# Autodesk Inventor assembly: FrameV4
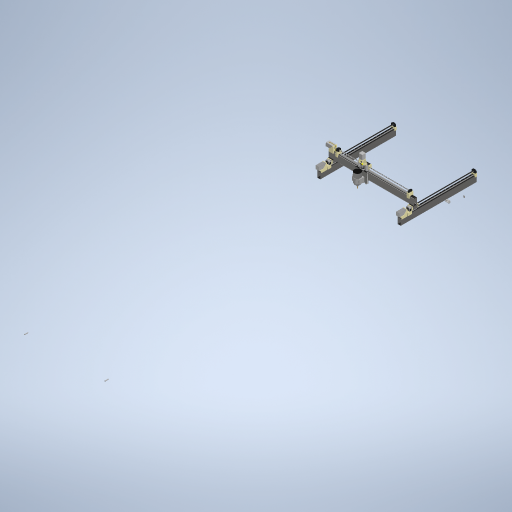
[picture p0: Inventor's stored thumbnail of the model, 512x512]
Saved by Autodesk Inventor 2023 (Build 270158000, 158)
## iProperties
Created: 2022-05-07
Part Number: FrameV4
Document SubType Name: Assembly
Designer: plebbb
Mass: 10930.1 g
Surface Area: 33660.3 cm^2
Volume: 10930.1 cm^3
Density: 1 g/cm^3
Author: plebbb
## Documents named in this file (27)
- C:\Users\a laptop\Desktop\CNC_Project\FrameV4.iam
- C:\Users\a laptop\Desktop\CNC_Project\Ballscrew_Assembly.iam
- C:\Users\a laptop\Desktop\CNC_Project\2x4_Tube.ipt
- C:\Users\a laptop\Desktop\CNC_Project\HGW20CC_Rail_800mm.ipt
- C:\Users\a laptop\Desktop\CNC_Project\BK10.ipt
- C:\Users\a laptop\Desktop\CNC_Project\BF10.ipt
- C:\Users\a laptop\Desktop\CNC_Project\Ballscrew_Assembly_1204.iam
- C:\Users\a laptop\Desktop\CNC_Project\SFU1204-500.ipt
- C:\Users\a laptop\Desktop\CNC_Project\BF10_Spacer.ipt
- C:\Users\a laptop\Desktop\CNC_Project\BK10_Spacer.ipt
- C:\Users\a laptop\Desktop\CNC_Project\2x3_L_Bracket.ipt
- C:\Users\a laptop\Desktop\CNC_Project\HGW20CC_Slider.ipt
- C:\Users\a laptop\Desktop\CNC_Project\HGW20CC_Rail_300mm.ipt
- C:\Users\a laptop\Desktop\CNC_Project\Z_PLATE.iam
- C:\Users\a laptop\Desktop\CNC_Project\SFU1204-300.ipt
- C:\Users\a laptop\Desktop\CNC_Project\Spindle.ipt
- C:\Users\a laptop\Desktop\CNC_Project\Drill_Bit.ipt
- C:\Users\a laptop\Desktop\CNC_Project\X_GANTRY.iam
- C:\Users\a laptop\Desktop\CNC_Project\Z_Gantry_Plate_Spaced.iam
- C:\Users\a laptop\Desktop\CNC_Project\Nema23.ipt
- C:\Users\a laptop\Desktop\CNC_Project\Nema23_Mount_short.ipt
- C:\Users\a laptop\Desktop\CNC_Project\SFU1204_Nut.ipt
- C:\Users\a laptop\Desktop\CNC_Project\DSG12H.ipt
- C:\Users\a laptop\Desktop\CNC_Project\Z_Motor_Holder.ipt
- C:\Users\a laptop\Desktop\CNC_Project\Nema23_Short.ipt
- C:\Users\a laptop\Desktop\CNC_Project\Xgantry_CableChain_bottom_connector.ipt
- C:\Users\a laptop\Desktop\CNC_Project\Xgantry_CableChain_top_connector.ipt
## Components (32 placed, 26 different names)
1. Ballscrew_Assembly:1 [sub-assembly] — Mate:7, Mate:8, Mate:11, Mate:84
2. Ballscrew_Assembly:2 [sub-assembly] — Mate:9, Mate:10, Mate:12, Mate:83, Mate:85, Mate:86
3. 2x4_Tube:1 — Mate:7, Mate:8, Mate:9, Mate:10, Mate:11, Mate:12, Flush:4, Mate:15, Mate:26, Mate:27, Mate:34, Mate:35, Flush:5, Mate:45
4. HGW20CC_Rail_800mm:1 — Flush:4, Mate:15, Mate:22, Mate:23, Mate:38, Flush:6, Flush:7
5. BK10:1 — Mate:40, Mate:41, Mate:42, Mate:43, Mate:44
6. BF10:1 — Mate:31, Mate:32, Mate:33, Mate:36
7. Ballscrew_Assembly_1204:1 [sub-assembly] — Mate:22, Mate:23, Mate:24, Mate:39, Mate:44, Mate:51, Mate:52
8. SFU1204-500:1 — Mate:24, Mate:36, Mate:43, Mate:89, Mate:90
9. BF10_Spacer:1 — Mate:31, Mate:32, Mate:33, Mate:34, Mate:35, Flush:5, Mate:38, Mate:39
10. BK10_Spacer:1 — Mate:26, Mate:27, Mate:40, Mate:41, Mate:42
11. 2x3_L_Bracket:1 — Mate:46, Mate:47, Mate:48
12. HGW20CC_Rail_800mm:2 — Flush:6, Mate:45, Mate:49, Mate:50, Flush:7
13. HGW20CC_Slider:1 — Mate:46, Mate:47, Mate:48, Mate:49, Mate:50
14. HGW20CC_Rail_300mm:1 — Flush:8, Angle:1, Angle:2, Flush:16, Flush:23
15. HGW20CC_Rail_300mm:2 — Flush:8, Angle:1, Mate:59, Mate:60
16. SFU1204-300:1 — Mate:66, Mate:99, Mate:100, Mate:101, Mate:105, Flush:24
17. Spindle:1 — Mate:75, Mate:76
18. Z_PLATE:1 [sub-assembly] — Mate:59, Mate:60, Flush:16, Mate:95, Flush:23
19. BK10:2 — Mate:66, Mate:97, Angle:4, Flush:24, Flush:25
20. Drill_Bit:1 — Mate:75, Mate:76
21. X_GANTRY:1 [sub-assembly] — Mate:80, Mate:81, Mate:82, Flush:21, Flush:22, Mate:83, Mate:85, Mate:86
22. X_GANTRY:2 [sub-assembly] — Flush:21, Flush:22, Mate:84
23. Z_Gantry_Plate_Spaced:1 [sub-assembly] — Mate:51, Mate:52, Angle:2, Mate:97, Mate:98, Angle:3, Flush:25, Flush:27
24. Nema23_Mount_short:1
25. Nema23:1 — Mate:89, Mate:90
26. SFU1204_Nut:1
27. DSG12H:1 — Mate:95
28. BF10:2 — Mate:98, Angle:3, Mate:99, Mate:100
29. Z_Motor_Holder:1 — Mate:101, Mate:102, Mate:103, Mate:104, Flush:27
30. Nema23_Short:1 — Mate:102, Mate:103, Mate:104, Mate:105, Angle:4
31. Xgantry_CableChain_bottom_connector:1
32. Xgantry_CableChain_top_connector:1
## Relationships (92: Mate 71, Flush 17, Angle 4)
- Mate:7: Ballscrew_Assembly:1 ↔ 2x4_Tube:1
- Mate:8: Ballscrew_Assembly:1 ↔ 2x4_Tube:1
- Mate:9: Ballscrew_Assembly:2 ↔ 2x4_Tube:1
- Mate:10: Ballscrew_Assembly:2 ↔ 2x4_Tube:1
- Mate:11: Ballscrew_Assembly:1 ↔ 2x4_Tube:1
- Mate:12: Ballscrew_Assembly:2 ↔ 2x4_Tube:1
- Flush:4 (15.4 mm): 2x4_Tube:1 ↔ HGW20CC_Rail_800mm:1
- Mate:15: 2x4_Tube:1 ↔ HGW20CC_Rail_800mm:1
- Mate:22: HGW20CC_Rail_800mm:1 ↔ Ballscrew_Assembly_1204:1
- Mate:23: HGW20CC_Rail_800mm:1 ↔ Ballscrew_Assembly_1204:1
- Mate:24: Ballscrew_Assembly_1204:1 ↔ SFU1204-500:1
- Mate:26: 2x4_Tube:1 ↔ BK10_Spacer:1
- Mate:27: 2x4_Tube:1 ↔ BK10_Spacer:1
- Mate:31: BF10:1 ↔ BF10_Spacer:1
- Mate:32: BF10:1 ↔ BF10_Spacer:1
- Mate:33: BF10:1 ↔ BF10_Spacer:1
- Mate:34: 2x4_Tube:1 ↔ BF10_Spacer:1
- Mate:35: 2x4_Tube:1 ↔ BF10_Spacer:1
- Mate:36: BF10:1 ↔ SFU1204-500:1
- Flush:5 (70 mm): 2x4_Tube:1 ↔ BF10_Spacer:1
- Mate:38: HGW20CC_Rail_800mm:1 ↔ BF10_Spacer:1
- Mate:39: Ballscrew_Assembly_1204:1 ↔ BF10_Spacer:1
- Mate:40: BK10:1 ↔ BK10_Spacer:1
- Mate:41: BK10:1 ↔ BK10_Spacer:1
- Mate:42: BK10:1 ↔ BK10_Spacer:1
- Mate:43: BK10:1 ↔ SFU1204-500:1
- Mate:44: BK10:1 ↔ Ballscrew_Assembly_1204:1
- Flush:6: HGW20CC_Rail_800mm:1 ↔ HGW20CC_Rail_800mm:2
- Mate:45: 2x4_Tube:1 ↔ HGW20CC_Rail_800mm:2
- Mate:46: 2x3_L_Bracket:1 ↔ HGW20CC_Slider:1
- Mate:47: 2x3_L_Bracket:1 ↔ HGW20CC_Slider:1
- Mate:48: 2x3_L_Bracket:1 ↔ HGW20CC_Slider:1
- Mate:49: HGW20CC_Rail_800mm:2 ↔ HGW20CC_Slider:1
- Mate:50: HGW20CC_Rail_800mm:2 ↔ HGW20CC_Slider:1
- Flush:7: HGW20CC_Rail_800mm:1 ↔ HGW20CC_Rail_800mm:2
- Mate:51: Ballscrew_Assembly_1204:1 ↔ Z_Gantry_Plate_Spaced:1
- Mate:52: Ballscrew_Assembly_1204:1 ↔ Z_Gantry_Plate_Spaced:1
- [Mate]: 2x3_L_Bracket:1 ↔ Z_Gantry_Plate_Spaced:1
- [Mate]: Ballscrew_Assembly_1204:1 ↔ Z_Gantry_Plate_Spaced:1
- Flush:8: HGW20CC_Rail_300mm:1 ↔ HGW20CC_Rail_300mm:2
- Angle:1 (0 deg): HGW20CC_Rail_300mm:1 ↔ HGW20CC_Rail_300mm:2
- Angle:2 (180 deg): HGW20CC_Rail_300mm:1 ↔ Z_Gantry_Plate_Spaced:1
- [Mate]: HGW20CC_Rail_300mm:1 ↔ Z_Gantry_Plate_Spaced:1
- [Mate]: HGW20CC_Rail_300mm:2 ↔ Z_Gantry_Plate_Spaced:1
- [Flush]: HGW20CC_Rail_300mm:1 ↔ Z_Gantry_Plate_Spaced:1
- [Flush]: HGW20CC_Rail_300mm:2 ↔ Z_Gantry_Plate_Spaced:1
- [Flush]: HGW20CC_Rail_300mm:2 ↔ Z_Gantry_Plate_Spaced:1
- Mate:59: HGW20CC_Rail_300mm:2 ↔ Z_PLATE:1
- Mate:60: HGW20CC_Rail_300mm:2 ↔ Z_PLATE:1
- Flush:16: HGW20CC_Rail_300mm:1 ↔ Z_PLATE:1
- [Mate]: SFU1204-300:1 ↔ SFU1204_Nut:1
- [Flush]: SFU1204-300:1 ↔ Z_Gantry_Plate_Spaced:1
- [Mate]: Spindle:1 ↔ Z_PLATE:1
- [Flush] (-20 mm): Spindle:1 ↔ Z_PLATE:1
- Mate:66: SFU1204-300:1 ↔ BK10:2
- Mate:75: Spindle:1 ↔ Drill_Bit:1
- Mate:76: Spindle:1 ↔ Drill_Bit:1
- [Mate] (10 mm): BK10:2 ↔ SFU1204_Nut:1
- Mate:80: X_GANTRY:1
- Mate:81: X_GANTRY:1
- Mate:82: X_GANTRY:1
- Flush:21: X_GANTRY:1 ↔ X_GANTRY:2
- Flush:22: X_GANTRY:1 ↔ X_GANTRY:2
- Mate:83: Ballscrew_Assembly:2 ↔ X_GANTRY:1
- Mate:84: Ballscrew_Assembly:1 ↔ X_GANTRY:2
- Mate:85: Ballscrew_Assembly:2 ↔ X_GANTRY:1
- Mate:86: Ballscrew_Assembly:2 ↔ X_GANTRY:1
- [Mate]: 2x4_Tube:1 ↔ Nema23_Mount_short:1
- [Mate] (0.25 mm): 2x4_Tube:1 ↔ Nema23_Mount_short:1
- Mate:89: SFU1204-500:1 ↔ Nema23:1
- Mate:90: SFU1204-500:1 ↔ Nema23:1
- [Mate]: Nema23_Mount_short:1 ↔ Nema23:1
- [Mate]: SFU1204_Nut:1 ↔ DSG12H:1
- [Mate]: SFU1204_Nut:1 ↔ DSG12H:1
- [Mate]: SFU1204_Nut:1 ↔ DSG12H:1
- Mate:95: Z_PLATE:1 ↔ DSG12H:1
- [Mate]: Z_PLATE:1 ↔ DSG12H:1
- Mate:97: BK10:2 ↔ Z_Gantry_Plate_Spaced:1
- Flush:23: HGW20CC_Rail_300mm:1 ↔ Z_PLATE:1
- Mate:98: Z_Gantry_Plate_Spaced:1 ↔ BF10:2
- Angle:3 (0 deg): Z_Gantry_Plate_Spaced:1 ↔ BF10:2
- Mate:99: SFU1204-300:1 ↔ BF10:2
- Mate:100: SFU1204-300:1 ↔ BF10:2
- Mate:101: SFU1204-300:1 ↔ Z_Motor_Holder:1
- Mate:102: Z_Motor_Holder:1 ↔ Nema23_Short:1
- Mate:103: Z_Motor_Holder:1 ↔ Nema23_Short:1
- Mate:104: Z_Motor_Holder:1 ↔ Nema23_Short:1
- Mate:105 (2 mm): SFU1204-300:1 ↔ Nema23_Short:1
- Angle:4 (0 deg): BK10:2 ↔ Nema23_Short:1
- Flush:24 (-22.75 mm): SFU1204-300:1 ↔ BK10:2
- Flush:25 (-4 mm): BK10:2 ↔ Z_Gantry_Plate_Spaced:1
- Flush:27 (0.15 mm): Z_Gantry_Plate_Spaced:1 ↔ Z_Motor_Holder:1
